# Autodesk Inventor assembly: square-50x15-x16
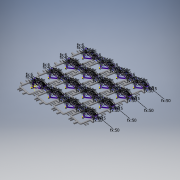
[picture p0: Inventor's stored thumbnail of the model, 180x180]
Saved by Autodesk Inventor 2016 (Build 200138000, 138)
## iProperties
Created: 2016-12-03
Part Number: square-50x15-x16
Document SubType Name: Assembly
Designer: Chris
Author: Chris
## Documents named in this file (2)
- F:\projects\161111 gleichseitige vielecke\square-50x15-x16.iam
- F:\projects\161111 gleichseitige vielecke\polygon.ipt
## Components (16 placed, 1 different names)
1. polygon:1
2. polygon:2
3. polygon:3
4. polygon:17
5. polygon:5
6. polygon:6
7. polygon:7
8. polygon:8
9. polygon:9
10. polygon:10
11. polygon:11
12. polygon:12
13. polygon:13
14. polygon:14
15. polygon:15
16. polygon:16
## Component patterns: (16 elements, first: polygon:1)
